# Autodesk Inventor assembly: Сборка1
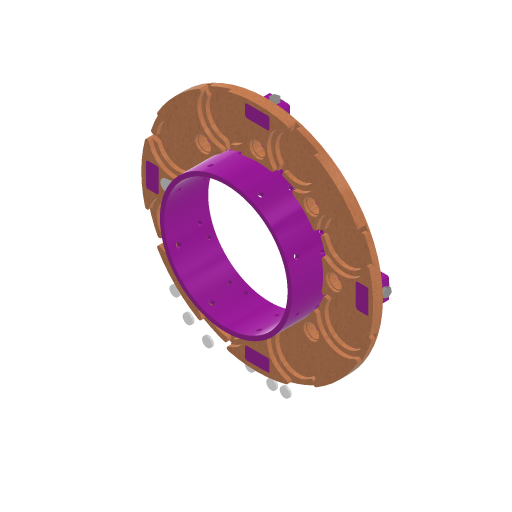
[picture p0: Inventor's stored thumbnail of the model, 512x512]
Saved by Autodesk Inventor 2023 (Build 270158000, 158)
## iProperties
Created: 2023-03-21
Part Number: Сборка1
Document SubType Name: Assembly
Designer: Admin
Author: Admin
## Documents named in this file (9)
- C:\Users\aleks\OneDrive\Рабочий стол\Хроматографический сортировщик\Детали\Сборка1.iam
- C:\Users\aleks\OneDrive\Рабочий стол\Хроматографический сортировщик\Детали\Барабан.ipt
- C:\Users\aleks\OneDrive\Рабочий стол\Хроматографический сортировщик\Детали\Короб для подшипника.ipt
- C:\Users\aleks\OneDrive\Рабочий стол\Хроматографический сортировщик\Детали\Покупные\Подшипник.ipt
- C:\Users\aleks\OneDrive\Рабочий стол\Хроматографический сортировщик\Детали\Покупные\Болт М5.ipt
- C:\Users\aleks\OneDrive\Рабочий стол\Хроматографический сортировщик\Детали\Покупные\Гайка М5 стопорная.ipt
- C:\Users\aleks\OneDrive\Рабочий стол\Хроматографический сортировщик\Детали\Покупные\Магнит.ipt
- C:\Users\aleks\OneDrive\Рабочий стол\Хроматографический сортировщик\Детали\Капсуль.ipt
- C:\Users\aleks\OneDrive\Рабочий стол\Хроматографический сортировщик\Детали\Покупные\Болт М5 круглый.ipt
## Components (28 placed, 8 different names)
1. Барабан:1 — Совмещение:9, Совмещение:10, Совмещение:11, Совмещение:12, Совмещение:13, Совмещение:14, Совмещение:15, Совмещение:16, Заподлицо:1, Заподлицо:2, Заподлицо:3, Заподлицо:4, Совмещение:57, Совмещение:58, Заподлицо:13, Совмещение:62, Совмещение:63
2. Короб для подшипника:1 — Совмещение:9, Совмещение:10, Заподлицо:4, Совмещение:17, Совмещение:21, Совмещение:27, Совмещение:32, Совмещение:34, Совмещение:37
3. Короб для подшипника:2 — Совмещение:11, Совмещение:12, Заподлицо:3, Совмещение:19, Совмещение:23, Совмещение:28, Совмещение:29, Совмещение:36, Совмещение:40
4. Короб для подшипника:3 — Совмещение:13, Совмещение:14, Заподлицо:2, Совмещение:20, Совмещение:24, Совмещение:25, Совмещение:30, Совмещение:35, Совмещение:39
5. Короб для подшипника:4 — Совмещение:15, Совмещение:16, Заподлицо:1, Совмещение:18, Совмещение:22, Совмещение:26, Совмещение:31, Совмещение:33, Совмещение:38
6. Подшипник:1 — Совмещение:18, Совмещение:22
7. Подшипник:2 — Совмещение:20, Совмещение:24
8. Подшипник:3 — Совмещение:19, Совмещение:23
9. Подшипник:4 — Совмещение:17, Совмещение:21
10. Болт М5:1 — Совмещение:25, Совмещение:35
11. Гайка М5 стопорная:1 — Совмещение:30, Совмещение:39
12. Болт М5:2 — Совмещение:26, Совмещение:33
13. Гайка М5 стопорная:2 — Совмещение:31, Совмещение:38
14. Болт М5:3 — Совмещение:27, Совмещение:34
15. Гайка М5 стопорная:3 — Совмещение:29, Совмещение:40
16. Болт М5:4 — Совмещение:28, Совмещение:36
17. Гайка М5 стопорная:4 — Совмещение:32, Совмещение:37
18. Магнит:1
19. Магнит:2
20. Магнит:3 — Совмещение:59, Заподлицо:14
21. Магнит:4
22. Магнит:5
23. Магнит:6
24. Магнит:7
25. Магнит:8
26. Капсуль:1 — Совмещение:57, Совмещение:58, Заподлицо:13, Совмещение:59, Заподлицо:14, Совмещение:60, Совмещение:61, Угол:1
27. Гайка М5 стопорная:5 — Совмещение:60, Совмещение:61, Угол:1
28. Болт М5 круглый:1 — Совмещение:62, Совмещение:63
## Relationships (46: Mate 39, Flush 6, Angle 1)
- Совмещение:9 [Mate]: Барабан:1 ↔ Короб для подшипника:1
- Совмещение:10 [Mate]: Барабан:1 ↔ Короб для подшипника:1
- Совмещение:11 [Mate]: Барабан:1 ↔ Короб для подшипника:2
- Совмещение:12 [Mate]: Барабан:1 ↔ Короб для подшипника:2
- Совмещение:13 [Mate]: Барабан:1 ↔ Короб для подшипника:3
- Совмещение:14 [Mate]: Барабан:1 ↔ Короб для подшипника:3
- Совмещение:15 [Mate]: Барабан:1 ↔ Короб для подшипника:4
- Совмещение:16 [Mate]: Барабан:1 ↔ Короб для подшипника:4
- Заподлицо:1 [Flush]: Барабан:1 ↔ Короб для подшипника:4
- Заподлицо:2 [Flush]: Барабан:1 ↔ Короб для подшипника:3
- Заподлицо:3 [Flush]: Барабан:1 ↔ Короб для подшипника:2
- Заподлицо:4 [Flush]: Барабан:1 ↔ Короб для подшипника:1
- Совмещение:17 [Mate]: Короб для подшипника:1 ↔ Подшипник:4
- Совмещение:18 [Mate]: Короб для подшипника:4 ↔ Подшипник:1
- Совмещение:19 [Mate]: Короб для подшипника:2 ↔ Подшипник:3
- Совмещение:20 [Mate]: Короб для подшипника:3 ↔ Подшипник:2
- Совмещение:21 [Mate] (0.5 mm): Короб для подшипника:1 ↔ Подшипник:4
- Совмещение:22 [Mate] (0.5 mm): Короб для подшипника:4 ↔ Подшипник:1
- Совмещение:23 [Mate] (0.5 mm): Короб для подшипника:2 ↔ Подшипник:3
- Совмещение:24 [Mate] (0.5 mm): Короб для подшипника:3 ↔ Подшипник:2
- Совмещение:25 [Mate]: Короб для подшипника:3 ↔ Болт М5:1
- Совмещение:26 [Mate]: Короб для подшипника:4 ↔ Болт М5:2
- Совмещение:27 [Mate]: Короб для подшипника:1 ↔ Болт М5:3
- Совмещение:28 [Mate]: Короб для подшипника:2 ↔ Болт М5:4
- Совмещение:29 [Mate]: Короб для подшипника:2 ↔ Гайка М5 стопорная:3
- Совмещение:30 [Mate]: Короб для подшипника:3 ↔ Гайка М5 стопорная:1
- Совмещение:31 [Mate]: Короб для подшипника:4 ↔ Гайка М5 стопорная:2
- Совмещение:32 [Mate]: Короб для подшипника:1 ↔ Гайка М5 стопорная:4
- Совмещение:33 [Mate]: Короб для подшипника:4 ↔ Болт М5:2
- Совмещение:34 [Mate]: Короб для подшипника:1 ↔ Болт М5:3
- Совмещение:35 [Mate]: Короб для подшипника:3 ↔ Болт М5:1
- Совмещение:36 [Mate]: Короб для подшипника:2 ↔ Болт М5:4
- Совмещение:37 [Mate]: Короб для подшипника:1 ↔ Гайка М5 стопорная:4
- Совмещение:38 [Mate]: Короб для подшипника:4 ↔ Гайка М5 стопорная:2
- Совмещение:39 [Mate]: Короб для подшипника:3 ↔ Гайка М5 стопорная:1
- Совмещение:40 [Mate]: Короб для подшипника:2 ↔ Гайка М5 стопорная:3
- Совмещение:57 [Mate]: Барабан:1 ↔ Капсуль:1
- Совмещение:58 [Mate]: Барабан:1 ↔ Капсуль:1
- Заподлицо:13 [Flush]: Барабан:1 ↔ Капсуль:1
- Совмещение:59 [Mate]: Магнит:3 ↔ Капсуль:1
- Заподлицо:14 [Flush]: Магнит:3 ↔ Капсуль:1
- Совмещение:60 [Mate]: Капсуль:1 ↔ Гайка М5 стопорная:5
- Совмещение:61 [Mate]: Капсуль:1 ↔ Гайка М5 стопорная:5
- Угол:1 [Angle] (0 deg): Капсуль:1 ↔ Гайка М5 стопорная:5
- Совмещение:62 [Mate]: Барабан:1 ↔ Болт М5 круглый:1
- Совмещение:63 [Mate]: Барабан:1 ↔ Болт М5 круглый:1
